# Autodesk Inventor assembly: Assembly2
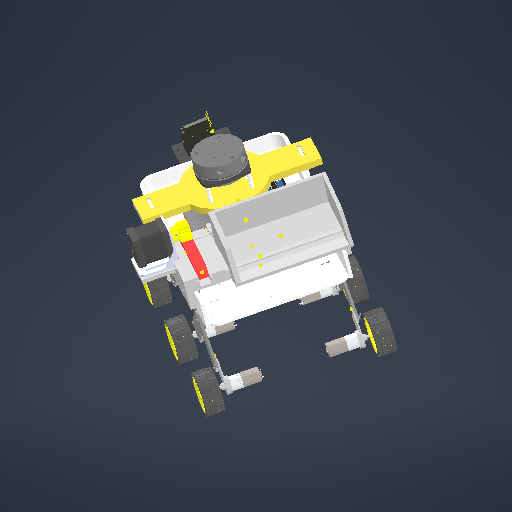
[picture p0: Inventor's stored thumbnail of the model, 512x512]
Saved by Autodesk Inventor 2027 (Build 310192000, 192)
## iProperties
Created: 2026-06-29
Part Number: Assembly2
Document SubType Name: Assembly
Designer: uchiha
Author: uchiha
## Documents named in this file (20)
- C:\Users\uchiha\Desktop\New folder\designdj\emmanuel-assembly.iam
- C:\Users\uchiha\Desktop\New folder\designdj\parts\rocker-bogie-mechanism-mars-rover-1.snapshot.9\assembly\bogie1.ipt
- C:\Users\uchiha\Desktop\New folder\designdj\parts\rocker-bogie-mechanism-mars-rover-1.snapshot.9\assembly\rocker1.ipt
- C:\Users\uchiha\Desktop\New folder\designdj\parts\rocker-bogie-mechanism-mars-rover-1.snapshot.9\assembly\platform.ipt
- C:\Users\uchiha\Desktop\New folder\designdj\parts\rocker-bogie-mechanism-mars-rover-1.snapshot.9\assembly\differantial.ipt
- C:\Users\uchiha\Desktop\New folder\designdj\parts\rocker-bogie-mechanism-mars-rover-1.snapshot.9\assembly\connector.ipt
- C:\Users\uchiha\Desktop\New folder\designdj\parts\rocker-bogie-mechanism-mars-rover-1.snapshot.9\assembly\L.ipt
- C:\Users\uchiha\Desktop\New folder\designdj\motorassembly.ipt
- C:\Users\uchiha\Desktop\New folder\designdj\parts\rocker-bogie-mechanism-mars-rover-1.snapshot.9\Assembly5.iam
- C:\Users\uchiha\Desktop\New folder\designdj\New folder\camera\motorbracket.ipt
- C:\Users\uchiha\Desktop\New folder\designdj\parts\20d-metal-gearmotors-3d-models\20d-metal-gearmotor-63-78\20d-metal-gearmotor-63-78.ipt
- C:\Users\uchiha\Desktop\New folder\designdj\rocker-bogie-mechanism-mars-rover-1.snapshot.9\assembly\wheel.ipt
- C:\Users\uchiha\Documents\Inventor\Content Center Files\R2027\en-US\AS 1110\AS 1110 - M3 x 6.ipt
- C:\Users\uchiha\Documents\Inventor\Content Center Files\R2027\en-US\AS 1110\AS 1110 - M2.5 x 6.ipt
- C:\Users\uchiha\Documents\Inventor\Content Center Files\R2027\en-US\AS 1110\AS 1110 - M2 x 6.ipt
- C:\Users\uchiha\Documents\Inventor\Content Center Files\R2027\en-US\AS 1110\AS 1110 - M1.6 x 6.ipt
- C:\Users\uchiha\Documents\Inventor\Content Center Files\R2027\en-US\ANSI B18.2.4.2M\ANSI B18.2.4.2M - M3x0.5 - 5.5.ipt
- C:\Users\uchiha\Documents\Inventor\Content Center Files\R2027\en-US\ANSI B18.2.4.2M\ANSI B18.2.4.2M - M3.5x0.6 - 6.ipt
- C:\Users\uchiha\Documents\Inventor\Content Center Files\R2027\en-US\AS 1112 (2)\AS 1112 - M1.6  Type 5.ipt
- C:\Users\uchiha\Documents\Inventor\Content Center Files\R2027\en-US\AS 1112 (2)\AS 1112 - M2.5  Type 5.ipt
## Components (117 placed, 19 different names)
1. bogie1:1 — Flush:4, Mate:51, Mate:52, Mate:53, Flush:5, Mate:54, Insert:13, Insert:28, Insert:29, Insert:30, Insert:31
2. rocker1:1 — Mate:48, Flush:3, Mate:49, Mate:50, Insert:14, Insert:15, Insert:16, Insert:34, Insert:35
3. platform:1 — Mate:56, Mate:57, Flush:6, Insert:7, Insert:8, Insert:9, Insert:10
4. platform:2 — Insert:36, Insert:37, Insert:38, Insert:39
5. rocker1:2 — Flush:2, Mate:32, Mate:33, Mate:34, Insert:17, Insert:18, Insert:19, Insert:76, Mate:82
6. bogie1:2 — Mate:10, Mate:11, Mate:15, Mate:17, Mate:18, Mate:19, Flush:1, Mate:25, Mate:26, Insert:24, Insert:25, Insert:26, Insert:27, Insert:32, Insert:33
7. differantial:1
8. connector:1 — Insert:40, Insert:41
9. connector:2 — Insert:11, Insert:12
10. L:1 — Mate:55, Mate:58, Mate:59
11. L:2 — Mate:60
12. L:3 — Insert:20, Insert:21, Insert:74, Insert:75
13. motorassembly:1
14. motorassembly:2
15. motorassembly:3
16. motorassembly:4 — Mate:10, Mate:11
17. Assembly5:1 [sub-assembly] — Mate:55, Mate:58, Mate:59, Mate:60, Insert:42, Insert:43, Insert:44, Insert:45, Insert:46, Insert:47, Insert:48, Insert:49, Insert:50, Insert:51, Insert:52, Insert:53, Insert:54, Insert:55, Insert:56, Insert:57, Insert:58, Insert:59, Insert:60, Insert:61, Insert:62, Insert:64, Insert:65, Insert:67, Insert:68, Insert:69
18. motorbracket:1 — Mate:12, Mate:13, Mate:14, Mate:15, Mate:16, Mate:17, Mate:18, Mate:19
19. 20d-metal-gearmotor-63-78:1 — Mate:12, Mate:13, Mate:14, Mate:16, Insert:4, Rotation:4
20. motorbracket:2 — Flush:1, Mate:25, Mate:26
21. 20d-metal-gearmotor-63-78:2 — Insert:3, Rotation:3
22. motorbracket:3 — Flush:2, Mate:32, Mate:33, Mate:34, Insert:22, Insert:23
23. 20d-metal-gearmotor-63-78:3 — Insert:2
24. motorbracket:4 — Mate:39, Mate:48, Flush:3, Mate:49, Mate:50
25. 20d-metal-gearmotor-63-78:4 — Mate:39, Insert:1, Rotation:1, Rotation:2
26. motorbracket:5 — Mate:53, Flush:5, Mate:54
27. 20d-metal-gearmotor-63-78:5 — Insert:5, Rotation:5, Rotation:6
28. motorbracket:6 — Flush:4, Mate:51, Mate:52
29. 20d-metal-gearmotor-63-78:6 — Insert:6, Rotation:7
30. L:4 — Mate:56, Mate:57, Flush:6, Insert:70, Insert:71, Insert:72, Insert:73
31. wheel:1 — Insert:2
32. wheel:2 — Insert:5, Rotation:5, Rotation:6
33. wheel:3 — Insert:1, Rotation:1, Rotation:2
34. wheel:4 — Insert:3, Rotation:3
35. wheel:5 — Insert:4, Rotation:4
36. wheel:7 — Insert:6, Rotation:7
37. AS 1110 - Metric M3 x 6:1 — Insert:7, Mate:71, Mate:72
38. AS 1110 - Metric M3 x 6:2 — Insert:8
39. AS 1110 - Metric M3 x 6:3 — Insert:9
40. AS 1110 - Metric M3 x 6:4 — Insert:10, Mate:69, Mate:70
41. AS 1110 - Metric M2.5 x 6:1 — Insert:11
42. AS 1110 - Metric M2.5 x 6:2 — Insert:12
43. AS 1110 - Metric M2.5 x 6:3 — Insert:13
44. AS 1110 - Metric M2.5 x 6:4 — Insert:14
45. AS 1110 - Metric M2.5 x 6:5 — Insert:15, Mate:83, Mate:84
46. AS 1110 - Metric M2.5 x 6:6 — Insert:16
47. AS 1110 - Metric M2.5 x 6:7 — Insert:17
48. AS 1110 - Metric M2.5 x 6:8 — Insert:18
49. AS 1110 - Metric M2.5 x 6:9 — Insert:19
50. AS 1110 - Metric M3 x 6:5 — Insert:20
51. AS 1110 - Metric M3 x 6:6 — Insert:21
52. AS 1110 - Metric M2 x 6:1 — Insert:22
53. AS 1110 - Metric M2.5 x 6:10 — Insert:23, Mate:81
54. AS 1110 - Metric M1.6 x 6:1 — Insert:24
55. AS 1110 - Metric M1.6 x 6:2 — Insert:25, Mate:73, Mate:74
56. AS 1110 - Metric M1.6 x 6:3 — Insert:26, Mate:75, Mate:76
57. AS 1110 - Metric M1.6 x 6:4 — Insert:27
58. AS 1110 - Metric M1.6 x 6:5 — Insert:28, Mate:77, Mate:78
59. AS 1110 - Metric M1.6 x 6:6 — Insert:29
60. AS 1110 - Metric M1.6 x 6:7 — Insert:30
61. AS 1110 - Metric M1.6 x 6:8 — Insert:31, Mate:79, Mate:80
62. AS 1110 - Metric M1.6 x 6:9 — Insert:32
63. AS 1110 - Metric M1.6 x 6:10 — Insert:33
64. AS 1110 - Metric M1.6 x 6:11 — Insert:34
65. AS 1110 - Metric M1.6 x 6:12 — Insert:35
66. AS 1110 - Metric M3 x 6:7 — Insert:36
67. AS 1110 - Metric M3 x 6:8 — Insert:37
68. AS 1110 - Metric M3 x 6:9 — Insert:38
69. AS 1110 - Metric M3 x 6:10 — Insert:39
70. AS 1110 - Metric M2.5 x 6:11 — Insert:40
71. AS 1110 - Metric M2.5 x 6:12 — Insert:41
72. AS 1110 - Metric M2.5 x 6:13 — Insert:42
73. AS 1110 - Metric M2.5 x 6:14 — Insert:43
74. AS 1110 - Metric M2.5 x 6:15 — Insert:44
75. AS 1110 - Metric M2.5 x 6:16 — Insert:45
76. AS 1110 - Metric M3 x 6:11 — Insert:46
77. AS 1110 - Metric M3 x 6:12 — Insert:47
78. AS 1110 - Metric M3 x 6:13 — Insert:48
79. AS 1110 - Metric M3 x 6:14 — Insert:49
80. AS 1110 - Metric M3 x 6:15 — Insert:50
81. AS 1110 - Metric M3 x 6:16 — Insert:51
82. AS 1110 - Metric M3 x 6:17 — Insert:52
83. AS 1110 - Metric M3 x 6:18 — Insert:53
84. AS 1110 - Metric M3 x 6:19 — Insert:54
85. AS 1110 - Metric M3 x 6:20 — Insert:55
86. AS 1110 - Metric M3 x 6:21 — Insert:56
87. AS 1110 - Metric M3 x 6:22 — Insert:57
88. AS 1110 - Metric M3 x 6:23 — Insert:58
89. AS 1110 - Metric M3 x 6:24 — Insert:59
90. AS 1110 - Metric M3 x 6:25 — Insert:60
91. AS 1110 - Metric M3 x 6:26 — Insert:61, Mate:61, Mate:62
92. AS 1110 - Metric M3 x 6:27 — Insert:62, Mate:63, Mate:64
93. AS 1110 - Metric M3 x 6:29 — Insert:64
94. AS 1110 - Metric M3 x 6:30 — Insert:65
95. AS 1110 - Metric M3 x 6:32 — Insert:67, Mate:65, Mate:66
96. AS 1110 - Metric M3 x 6:33 — Insert:68, Mate:67, Mate:68
97. AS 1110 - Metric M3 x 6:34 — Insert:69
98. ANSI B18.2.4.2M M3x0.5:1 — Mate:61, Mate:62
99. ANSI B18.2.4.2M M3x0.5:2 — Mate:63, Mate:64
100. ANSI B18.2.4.2M M3x0.5:3 — Mate:65, Mate:66
101. ANSI B18.2.4.2M M3x0.5:4 — Mate:67, Mate:68
102. ANSI B18.2.4.2M M3x0.5:5 — Mate:69, Mate:70
103. ANSI B18.2.4.2M M3x0.5:6 — Mate:71, Mate:72
104. ANSI B18.2.4.2M M3.5x0.6:1 — Insert:70
105. ANSI B18.2.4.2M M3.5x0.6:2 — Insert:71
106. ANSI B18.2.4.2M M3.5x0.6:3 — Insert:72
107. ANSI B18.2.4.2M M3.5x0.6:4 — Insert:73
108. ANSI B18.2.4.2M M3.5x0.6:5 — Insert:74
109. ANSI B18.2.4.2M M3.5x0.6:6 — Insert:75
110. AS 1112 (2) - Metric M1.6  Type 5:1 — Mate:73, Mate:74
111. AS 1112 (2) - Metric M1.6  Type 5:2 — Mate:75, Mate:76
112. AS 1112 (2) - Metric M1.6  Type 5:3 — Mate:77, Mate:78
113. AS 1112 (2) - Metric M1.6  Type 5:4 — Mate:79, Mate:80
114. AS 1112 (2) - Metric M1.6  Type 5:5 — Insert:76
115. AS 1112 (2) - Metric M2.5  Type 5:1 — Mate:81, Mate:82
116. AS 1112 (2) - Metric M2.5  Type 5:2 — Mate:83, Mate:84
117. AS 1110 - Metric M2.5 x 6:19
## Relationships (160: Insert 74, Mate 73, RelateRotation 7, Flush 6)
- Mate:10: bogie1:2 ↔ motorassembly:4
- Mate:11: bogie1:2 ↔ motorassembly:4
- Mate:12: motorbracket:1 ↔ 20d-metal-gearmotor-63-78:1
- Mate:13: motorbracket:1 ↔ 20d-metal-gearmotor-63-78:1
- Mate:14: motorbracket:1 ↔ 20d-metal-gearmotor-63-78:1
- Mate:15: bogie1:2 ↔ motorbracket:1
- Mate:16: motorbracket:1 ↔ 20d-metal-gearmotor-63-78:1
- Mate:17: bogie1:2 ↔ motorbracket:1
- Mate:18: bogie1:2 ↔ motorbracket:1
- Mate:19: bogie1:2 ↔ motorbracket:1
- [Mate]: motorbracket:2 ↔ 20d-metal-gearmotor-63-78:2
- [Mate]: motorbracket:2 ↔ 20d-metal-gearmotor-63-78:2
- [Mate]: motorbracket:2 ↔ 20d-metal-gearmotor-63-78:2
- [Mate]: motorbracket:2 ↔ 20d-metal-gearmotor-63-78:2
- Flush:1: bogie1:2 ↔ motorbracket:2
- Mate:25: bogie1:2 ↔ motorbracket:2
- Mate:26: bogie1:2 ↔ motorbracket:2
- [Mate]: motorbracket:3 ↔ 20d-metal-gearmotor-63-78:3
- [Mate]: motorbracket:3 ↔ 20d-metal-gearmotor-63-78:3
- [Mate]: motorbracket:3 ↔ 20d-metal-gearmotor-63-78:3
- [Mate]: motorbracket:3 ↔ 20d-metal-gearmotor-63-78:3
- Flush:2: rocker1:2 ↔ motorbracket:3
- Mate:32: rocker1:2 ↔ motorbracket:3
- Mate:33: rocker1:2 ↔ motorbracket:3
- Mate:34: rocker1:2 ↔ motorbracket:3
- [Mate]: motorbracket:4 ↔ 20d-metal-gearmotor-63-78:4
- [Mate]: motorbracket:4 ↔ 20d-metal-gearmotor-63-78:4
- [Mate]: motorbracket:4 ↔ 20d-metal-gearmotor-63-78:4
- [Mate]: motorbracket:4 ↔ 20d-metal-gearmotor-63-78:4
- Mate:39: motorbracket:4 ↔ 20d-metal-gearmotor-63-78:4
- [Mate]: motorbracket:5 ↔ 20d-metal-gearmotor-63-78:5
- [Mate]: motorbracket:5 ↔ 20d-metal-gearmotor-63-78:5
- [Mate]: motorbracket:5 ↔ 20d-metal-gearmotor-63-78:5
- [Mate]: motorbracket:5 ↔ 20d-metal-gearmotor-63-78:5
- [Mate]: motorbracket:6 ↔ 20d-metal-gearmotor-63-78:6
- [Mate]: motorbracket:6 ↔ 20d-metal-gearmotor-63-78:6
- [Mate]: motorbracket:6 ↔ 20d-metal-gearmotor-63-78:6
- [Mate]: motorbracket:6 ↔ 20d-metal-gearmotor-63-78:6
- Mate:48: rocker1:1 ↔ motorbracket:4
- Flush:3: rocker1:1 ↔ motorbracket:4
- Mate:49: rocker1:1 ↔ motorbracket:4
- Mate:50: rocker1:1 ↔ motorbracket:4
- Flush:4: bogie1:1 ↔ motorbracket:6
- Mate:51: bogie1:1 ↔ motorbracket:6
- Mate:52: bogie1:1 ↔ motorbracket:6
- Mate:53: bogie1:1 ↔ motorbracket:5
- Flush:5: bogie1:1 ↔ motorbracket:5
- Mate:54: bogie1:1 ↔ motorbracket:5
- Mate:55: L:1 ↔ Assembly5:1
- Mate:56: platform:1 ↔ L:4
- Mate:57: platform:1 ↔ L:4
- Flush:6: platform:1 ↔ L:4
- Mate:58: L:1 ↔ Assembly5:1
- Mate:59: L:1 ↔ Assembly5:1
- Mate:60: L:2 ↔ Assembly5:1
- Insert:1 (-5 mm): 20d-metal-gearmotor-63-78:4 ↔ wheel:3
- Rotation:1 [RelateRotation] (0.571 ul): 20d-metal-gearmotor-63-78:4 ↔ wheel:3
- Rotation:2 [RelateRotation] (0.571 ul): 20d-metal-gearmotor-63-78:4 ↔ wheel:3
- Insert:2 (-5 mm): 20d-metal-gearmotor-63-78:3 ↔ wheel:1
- Insert:3 (-5 mm): 20d-metal-gearmotor-63-78:2 ↔ wheel:4
- Rotation:3 [RelateRotation] (0.8 ul): 20d-metal-gearmotor-63-78:2 ↔ wheel:4
- Insert:4 (-4 mm): 20d-metal-gearmotor-63-78:1 ↔ wheel:5
- Rotation:4 [RelateRotation] (0.571 ul): 20d-metal-gearmotor-63-78:1 ↔ wheel:5
- Insert:5 (-5 mm): 20d-metal-gearmotor-63-78:5 ↔ wheel:2
- Rotation:5 [RelateRotation] (1 ul): 20d-metal-gearmotor-63-78:5 ↔ wheel:2
- Rotation:6 [RelateRotation] (0.571 ul): 20d-metal-gearmotor-63-78:5 ↔ wheel:2
- Insert:6 (-5 mm): 20d-metal-gearmotor-63-78:6 ↔ wheel:7
- Rotation:7 [RelateRotation] (1.75 ul): 20d-metal-gearmotor-63-78:6 ↔ wheel:7
- Insert:7: platform:1 ↔ AS 1110 - Metric M3 x 6:1
- Insert:8: platform:1 ↔ AS 1110 - Metric M3 x 6:2
- Insert:9: platform:1 ↔ AS 1110 - Metric M3 x 6:3
- Insert:10: platform:1 ↔ AS 1110 - Metric M3 x 6:4
- Insert:11: connector:2 ↔ AS 1110 - Metric M2.5 x 6:1
- Insert:12: connector:2 ↔ AS 1110 - Metric M2.5 x 6:2
- Insert:13: bogie1:1 ↔ AS 1110 - Metric M2.5 x 6:3
- Insert:14: rocker1:1 ↔ AS 1110 - Metric M2.5 x 6:4
- Insert:15: rocker1:1 ↔ AS 1110 - Metric M2.5 x 6:5
- Insert:16: rocker1:1 ↔ AS 1110 - Metric M2.5 x 6:6
- Insert:17: rocker1:2 ↔ AS 1110 - Metric M2.5 x 6:7
- Insert:18: rocker1:2 ↔ AS 1110 - Metric M2.5 x 6:8
- Insert:19: rocker1:2 ↔ AS 1110 - Metric M2.5 x 6:9
- Insert:20: L:3 ↔ AS 1110 - Metric M3 x 6:5
- Insert:21: L:3 ↔ AS 1110 - Metric M3 x 6:6
- Insert:22: motorbracket:3 ↔ AS 1110 - Metric M2 x 6:1
- Insert:23: motorbracket:3 ↔ AS 1110 - Metric M2.5 x 6:10
- Insert:24: bogie1:2 ↔ AS 1110 - Metric M1.6 x 6:1
- Insert:25: bogie1:2 ↔ AS 1110 - Metric M1.6 x 6:2
- Insert:26: bogie1:2 ↔ AS 1110 - Metric M1.6 x 6:3
- Insert:27: bogie1:2 ↔ AS 1110 - Metric M1.6 x 6:4
- Insert:28: bogie1:1 ↔ AS 1110 - Metric M1.6 x 6:5
- Insert:29: bogie1:1 ↔ AS 1110 - Metric M1.6 x 6:6
- Insert:30: bogie1:1 ↔ AS 1110 - Metric M1.6 x 6:7
- Insert:31: bogie1:1 ↔ AS 1110 - Metric M1.6 x 6:8
- Insert:32: bogie1:2 ↔ AS 1110 - Metric M1.6 x 6:9
- Insert:33: bogie1:2 ↔ AS 1110 - Metric M1.6 x 6:10
- Insert:34: rocker1:1 ↔ AS 1110 - Metric M1.6 x 6:11
- Insert:35: rocker1:1 ↔ AS 1110 - Metric M1.6 x 6:12
- Insert:36: platform:2 ↔ AS 1110 - Metric M3 x 6:7
- Insert:37: platform:2 ↔ AS 1110 - Metric M3 x 6:8
- Insert:38: platform:2 ↔ AS 1110 - Metric M3 x 6:9
- Insert:39: platform:2 ↔ AS 1110 - Metric M3 x 6:10
- Insert:40: connector:1 ↔ AS 1110 - Metric M2.5 x 6:11
- Insert:41: connector:1 ↔ AS 1110 - Metric M2.5 x 6:12
- Insert:42: Assembly5:1 ↔ AS 1110 - Metric M2.5 x 6:13
- Insert:43: Assembly5:1 ↔ AS 1110 - Metric M2.5 x 6:14
- Insert:44: Assembly5:1 ↔ AS 1110 - Metric M2.5 x 6:15
- Insert:45: Assembly5:1 ↔ AS 1110 - Metric M2.5 x 6:16
- Insert:46: Assembly5:1 ↔ AS 1110 - Metric M3 x 6:11
- Insert:47: Assembly5:1 ↔ AS 1110 - Metric M3 x 6:12
- Insert:48: Assembly5:1 ↔ AS 1110 - Metric M3 x 6:13
- Insert:49: Assembly5:1 ↔ AS 1110 - Metric M3 x 6:14
- Insert:50: Assembly5:1 ↔ AS 1110 - Metric M3 x 6:15
- Insert:51: Assembly5:1 ↔ AS 1110 - Metric M3 x 6:16
- Insert:52: Assembly5:1 ↔ AS 1110 - Metric M3 x 6:17
- Insert:53: Assembly5:1 ↔ AS 1110 - Metric M3 x 6:18
- Insert:54: Assembly5:1 ↔ AS 1110 - Metric M3 x 6:19
- Insert:55: Assembly5:1 ↔ AS 1110 - Metric M3 x 6:20
- Insert:56: Assembly5:1 ↔ AS 1110 - Metric M3 x 6:21
- Insert:57: Assembly5:1 ↔ AS 1110 - Metric M3 x 6:22
- Insert:58: Assembly5:1 ↔ AS 1110 - Metric M3 x 6:23
- Insert:59: Assembly5:1 ↔ AS 1110 - Metric M3 x 6:24
- Insert:60: Assembly5:1 ↔ AS 1110 - Metric M3 x 6:25
- Insert:61: Assembly5:1 ↔ AS 1110 - Metric M3 x 6:26
- Insert:62: Assembly5:1 ↔ AS 1110 - Metric M3 x 6:27
- Insert:64: Assembly5:1 ↔ AS 1110 - Metric M3 x 6:29
- Insert:65: Assembly5:1 ↔ AS 1110 - Metric M3 x 6:30
- Insert:67: Assembly5:1 ↔ AS 1110 - Metric M3 x 6:32
- Insert:68: Assembly5:1 ↔ AS 1110 - Metric M3 x 6:33
- Insert:69: Assembly5:1 ↔ AS 1110 - Metric M3 x 6:34
- Mate:61: AS 1110 - Metric M3 x 6:26 ↔ ANSI B18.2.4.2M M3x0.5:1
- Mate:62: AS 1110 - Metric M3 x 6:26 ↔ ANSI B18.2.4.2M M3x0.5:1
- Mate:63: AS 1110 - Metric M3 x 6:27 ↔ ANSI B18.2.4.2M M3x0.5:2
- Mate:64: AS 1110 - Metric M3 x 6:27 ↔ ANSI B18.2.4.2M M3x0.5:2
- Mate:65: AS 1110 - Metric M3 x 6:32 ↔ ANSI B18.2.4.2M M3x0.5:3
- Mate:66: AS 1110 - Metric M3 x 6:32 ↔ ANSI B18.2.4.2M M3x0.5:3
- Mate:67: AS 1110 - Metric M3 x 6:33 ↔ ANSI B18.2.4.2M M3x0.5:4
- Mate:68: AS 1110 - Metric M3 x 6:33 ↔ ANSI B18.2.4.2M M3x0.5:4
- Mate:69: AS 1110 - Metric M3 x 6:4 ↔ ANSI B18.2.4.2M M3x0.5:5
- Mate:70: AS 1110 - Metric M3 x 6:4 ↔ ANSI B18.2.4.2M M3x0.5:5
- Mate:71: AS 1110 - Metric M3 x 6:1 ↔ ANSI B18.2.4.2M M3x0.5:6
- Mate:72: AS 1110 - Metric M3 x 6:1 ↔ ANSI B18.2.4.2M M3x0.5:6
- Insert:70: L:4 ↔ ANSI B18.2.4.2M M3.5x0.6:1
- Insert:71: L:4 ↔ ANSI B18.2.4.2M M3.5x0.6:2
- Insert:72: L:4 ↔ ANSI B18.2.4.2M M3.5x0.6:3
- Insert:73: L:4 ↔ ANSI B18.2.4.2M M3.5x0.6:4
- Insert:74: L:3 ↔ ANSI B18.2.4.2M M3.5x0.6:5
- Insert:75: L:3 ↔ ANSI B18.2.4.2M M3.5x0.6:6
- Mate:73: AS 1110 - Metric M1.6 x 6:2 ↔ AS 1112 (2) - Metric M1.6  Type 5:1
- Mate:74: AS 1110 - Metric M1.6 x 6:2 ↔ AS 1112 (2) - Metric M1.6  Type 5:1
- Mate:75: AS 1110 - Metric M1.6 x 6:3 ↔ AS 1112 (2) - Metric M1.6  Type 5:2
- Mate:76: AS 1110 - Metric M1.6 x 6:3 ↔ AS 1112 (2) - Metric M1.6  Type 5:2
- Mate:77: AS 1110 - Metric M1.6 x 6:5 ↔ AS 1112 (2) - Metric M1.6  Type 5:3
- Mate:78: AS 1110 - Metric M1.6 x 6:5 ↔ AS 1112 (2) - Metric M1.6  Type 5:3
- Mate:79: AS 1110 - Metric M1.6 x 6:8 ↔ AS 1112 (2) - Metric M1.6  Type 5:4
- Mate:80: AS 1110 - Metric M1.6 x 6:8 ↔ AS 1112 (2) - Metric M1.6  Type 5:4
- Insert:76: rocker1:2 ↔ AS 1112 (2) - Metric M1.6  Type 5:5
- Mate:81: AS 1110 - Metric M2.5 x 6:10 ↔ AS 1112 (2) - Metric M2.5  Type 5:1
- Mate:82: rocker1:2 ↔ AS 1112 (2) - Metric M2.5  Type 5:1
- Mate:83: AS 1110 - Metric M2.5 x 6:5 ↔ AS 1112 (2) - Metric M2.5  Type 5:2
- Mate:84: AS 1110 - Metric M2.5 x 6:5 ↔ AS 1112 (2) - Metric M2.5  Type 5:2
## Named parameters: d43_d39 = 0 mm, d47_d35 = 0 mm, d48_d36 = 0 mm, d49_d37 = 0 mm, d54_d39 = 0 mm, d58_d35 = 0 mm, d59_d36 = 0 mm, d60_d37 = 0 mm, d66_d54_d39 = 0 mm, d67_d58_d35 = 0 mm, d68_d59_d36 = 0 mm, d69_d60_d37 = 0 mm, d71_d54_d39 = 0 mm, d72_d58_d35 = 0 mm, d73_d59_d36 = 0 mm, d74_d60_d37 = 0 mm, d75_d54_d39 = 0 mm, d76_d58_d35 = 0 mm, d77_d59_d36 = 0 mm, d78_d60_d37 = 0 mm
